# Autodesk Inventor assembly: ASY Лестница перила
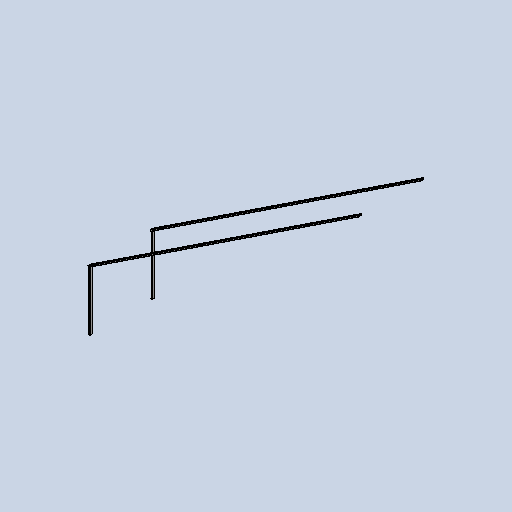
[picture p0: Inventor's stored thumbnail of the model, 512x512]
Saved by Autodesk Inventor 2025 (Build 290162010, 162A)
## iProperties
Created: 2025-01-21
Part Number: ASY Лестница перила
Document SubType Name: Assembly
Designer: pokla
Author: pokla
## Documents named in this file (3)
- C:\Users\pokla\Documents\Inventor\NDM-VOS_powder_hopper\ASY Лестница перила.iam
- C:\Users\pokla\Documents\Inventor\NDM-VOS_powder_hopper\ISO 4019 - 40x20x2 - 950.ipt
- C:\Users\pokla\Documents\Inventor\NDM-VOS_powder_hopper\ISO 4019 - 40x20x2 - 3000.ipt
## Components (4 placed, 2 different names)
1. ISO 4019 - 40x20x2 - 950:1
2. ISO 4019 - 40x20x2 - 950:2
3. ISO 4019 - 40x20x2 - 3000:1
4. ISO 4019 - 40x20x2 - 3000:2
## Relationships (2: WeldJoint 2)
- [WeldJoint]: ISO 4019 - 40x20x2 - 950:1 ↔ ISO 4019 - 40x20x2 - 3000:1
- [WeldJoint]: ISO 4019 - 40x20x2 - 950:2 ↔ ISO 4019 - 40x20x2 - 3000:2
